# Autodesk Inventor assembly: A2017_T3_03
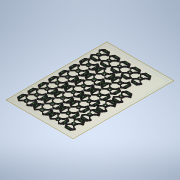
[picture p0: Inventor's stored thumbnail of the model, 180x180]
Saved by Autodesk Inventor 2022 (Build 260153000, 153)
## iProperties
Created: 2022-09-28
Part Number: A2017_T3_03
Document SubType Name: Assembly
Designer: Masato
Author: Masato
## Documents named in this file (3)
- C:\Users\6343y\ドキュメント\Inventor\SUSTAINA-OP\Cam\A2017_T3\A2017_T3_03.iam
- C:\Users\6343y\ドキュメント\Inventor\SUSTAINA-OP\Cam\DisposableBoard.ipt
- C:\Users\6343y\ドキュメント\Inventor\SUSTAINA-OP\LowerBody\Leg_joint\Leg_joint_roll_frame.ipt
## Components (31 placed, 2 different names)
1. DisposableBoard:1 — フラッシュ:1, フラッシュ:2, フラッシュ:3, フラッシュ:4, Tangent:1, Flush:5, 正接:2, 正接:4, フラッシュ:6
2. Leg_joint_roll_frame:2 — Tangent:1, Flush:5, Mate:5
3. Leg_joint_roll_frame:3
4. Leg_joint_roll_frame:4 — 正接:5
5. Leg_joint_roll_frame:5
6. Leg_joint_roll_frame:6
7. Leg_joint_roll_frame:7
8. Leg_joint_roll_frame:8
9. Leg_joint_roll_frame:9
10. Leg_joint_roll_frame:10
11. Leg_joint_roll_frame:11
12. Leg_joint_roll_frame:12
13. Leg_joint_roll_frame:13
14. Leg_joint_roll_frame:14
15. Leg_joint_roll_frame:15
16. Leg_joint_roll_frame:16
17. Leg_joint_roll_frame:17
18. Leg_joint_roll_frame:18
19. Leg_joint_roll_frame:19
20. Leg_joint_roll_frame:20 — 正接:3
21. Leg_joint_roll_frame:21
22. Leg_joint_roll_frame:22
23. Leg_joint_roll_frame:23 — メイト:6, 正接:2, 正接:3, 正接:4
24. Leg_joint_roll_frame:24
25. Leg_joint_roll_frame:25
26. Leg_joint_roll_frame:26
27. Leg_joint_roll_frame:27
28. Leg_joint_roll_frame:28 — メイト:7, フラッシュ:6, 正接:5
29. Leg_joint_roll_frame:29
30. Leg_joint_roll_frame:30
31. Leg_joint_roll_frame:31
## Component patterns: (21 elements, first: Leg_joint_roll_frame:2), (5 elements, first: Leg_joint_roll_frame:23), (4 elements, first: Leg_joint_roll_frame:28)
## Relationships (14: Flush 6, Tangent 5, Mate 3)
- フラッシュ:1 [Flush]: DisposableBoard:1
- フラッシュ:2 [Flush]: DisposableBoard:1
- フラッシュ:3 [Flush]: DisposableBoard:1
- フラッシュ:4 [Flush]: DisposableBoard:1
- Tangent:1 (2 mm): DisposableBoard:1 ↔ Leg_joint_roll_frame:2
- Flush:5 (-2 mm): DisposableBoard:1 ↔ Leg_joint_roll_frame:2
- Mate:5: Leg_joint_roll_frame:2
- メイト:6 [Mate]: Leg_joint_roll_frame:23
- 正接:2 [Tangent] (2.1 mm): DisposableBoard:1 ↔ Leg_joint_roll_frame:23
- 正接:3 [Tangent] (2.1 mm): Leg_joint_roll_frame:20 ↔ Leg_joint_roll_frame:23
- 正接:4 [Tangent] (2.1 mm): DisposableBoard:1 ↔ Leg_joint_roll_frame:23
- メイト:7 [Mate]: Leg_joint_roll_frame:28
- フラッシュ:6 [Flush] (2.1 mm): DisposableBoard:1 ↔ Leg_joint_roll_frame:28
- 正接:5 [Tangent] (2.1 mm): Leg_joint_roll_frame:4 ↔ Leg_joint_roll_frame:28
